# Autodesk Inventor assembly: ASY TZS 1662 FDS way 2
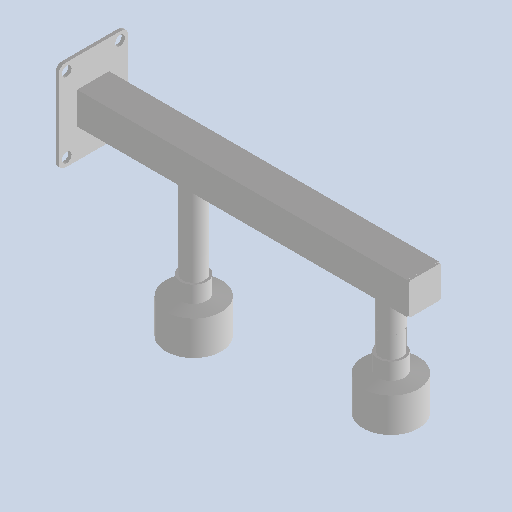
[picture p0: Inventor's stored thumbnail of the model, 512x512]
Saved by Autodesk Inventor 2025 (Build 290162010, 162A)
## iProperties
Created: 2025-07-02
Part Number: ASY TZS 1662 FDS way 2
Document SubType Name: Assembly
Designer: admin
Author: user
## Documents named in this file (8)
- C:\Users\pokla\Documents\Inventor\TZS-Tazovskiy\Filter D940\FDS 940\ASY TZS 1662 FDS way 2.iam
- C:\Users\pokla\Documents\Inventor\TZS-Tazovskiy\Filter D940\FDS 940\TZS 1662 FDS 940 way tube 2.ipt
- C:\Users\pokla\Documents\Inventor\TZS-Tazovskiy\Filter D940\FDS 940\TZS dummy filter element_940.ipt
- C:\Users\pokla\Documents\Inventor\TZS-Tazovskiy\Filter D940\FDS 940\TZS dummy pipe nippel_940.ipt
- C:\Users\pokla\Documents\Inventor\TZS-Tazovskiy\Filter D940\FDS 940\TZS 1686 FDS 940 way tube 6.ipt
- C:\Users\pokla\Documents\Inventor\TZS-Tazovskiy\Filter D940\FDS 940\TZS 1687 FDS 940 way tube 7.ipt
- C:\Users\pokla\Documents\Inventor\TZS-Tazovskiy\Filter D940\FDS 940\TZS 1669 FDS 940 FLANGE 3.ipt
- C:\Users\pokla\Documents\Inventor\TZS-Tazovskiy\Filter D940\FDS 940\TZS 1666 FDS 940 CUP 1.ipt
## Components (9 placed, 7 different names)
1. TZS 1662 FDS 940 way tube 2.ipt:1 — Rigid:5, Rigid:8, Rigid:9, Rigid:10
2. TZS 1686 FDS 940 way tube 6.ipt:1 — Rigid:5, Rigid:4
3. TZS dummy filter element_940.ipt:1 — Rigid:3
4. TZS dummy pipe nippel_940.ipt:1 — Rigid:4, Rigid:3
5. TZS 1687 FDS 940 way tube 7.ipt:1 — Rigid:8, Rigid:7
6. TZS dummy filter element_940.ipt:2 — Rigid:6
7. TZS dummy pipe nippel_940.ipt:2 — Rigid:7, Rigid:6
8. TZS 1669 FDS 940 FLANGE 3.ipt:1 — Rigid:9
9. TZS 1666 FDS 940 CUP 1.ipt:1 — Rigid:10
## Relationships (8: WeldJoint 8)
- Rigid:5 [WeldJoint]: TZS 1662 FDS 940 way tube 2.ipt:1 ↔ TZS 1686 FDS 940 way tube 6.ipt:1
- Rigid:4 [WeldJoint]: TZS 1686 FDS 940 way tube 6.ipt:1 ↔ TZS dummy pipe nippel_940.ipt:1
- Rigid:3 [WeldJoint]: TZS dummy filter element_940.ipt:1 ↔ TZS dummy pipe nippel_940.ipt:1
- Rigid:8 [WeldJoint]: TZS 1662 FDS 940 way tube 2.ipt:1 ↔ TZS 1687 FDS 940 way tube 7.ipt:1
- Rigid:7 [WeldJoint]: TZS 1687 FDS 940 way tube 7.ipt:1 ↔ TZS dummy pipe nippel_940.ipt:2
- Rigid:6 [WeldJoint]: TZS dummy filter element_940.ipt:2 ↔ TZS dummy pipe nippel_940.ipt:2
- Rigid:9 [WeldJoint] (-3 mm): TZS 1662 FDS 940 way tube 2.ipt:1 ↔ TZS 1669 FDS 940 FLANGE 3.ipt:1
- Rigid:10 [WeldJoint]: TZS 1662 FDS 940 way tube 2.ipt:1 ↔ TZS 1666 FDS 940 CUP 1.ipt:1
